# Autodesk Inventor assembly: BBM Staging Plate Assembly
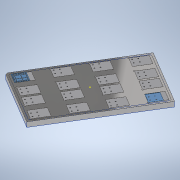
[picture p0: Inventor's stored thumbnail of the model, 180x180]
Saved by Autodesk Inventor 2022 (Build 260153000, 153)
## iProperties
Created: 2021-01-11
Part Number: BBM Staging Plate Assembly
Document SubType Name: Assembly
Designer: caleb
Author: caleb
## Documents named in this file (5)
- C:\Users\Caleb\Desktop\nebraska-silicon-lab\Hardware\ETL\Module Assembly\BBM Staging Plate - V2\BBM Staging Plate Assembly - V2.iam
- C:\Users\Caleb\Desktop\nebraska-silicon-lab\Hardware\ETL\Module Assembly\BBM Staging Plate - V2\BBM Staging Plate - V2.ipt
- C:\Users\Caleb\Desktop\nebraska-silicon-lab\Hardware\ETL\Module Assembly\BBM Staging Plate - V2\BBM Staging Plate Stencil - V2.ipt
- C:\Users\Caleb\Desktop\nebraska-silicon-lab\Hardware\ETL\Module Assembly\BBM Staging Plate - V2\Plastic Inlay.ipt
- C:\Users\Caleb\Desktop\nebraska-silicon-lab\Hardware\ETL\Module Assembly\BBM Staging Plate - V2\F10112319--_1-MODULE_ CMS2 ETL_ PIXEL SENSOR READOUT CHIP.ipt
## Components (5 placed, 4 different names)
1. BBM Staging Plate - V2:1 — Flush:1, Flush:2, Mate:1, Mate:2, Mate:3, Mate:4
2. BBM Staging Plate Stencil - V2:1 — Flush:1, Flush:2, Mate:1, Mate:6, Mate:7, Mate:9, Mate:10
3. Plastic Inlay:1 — Mate:2, Mate:3, Mate:4, Mate:5, Mate:8
4. F10112319--_1-MODULE_ CMS2 ETL_ PIXEL SENSOR READOUT CHIP:1 — Mate:5, Mate:6, Mate:7
5. F10112319--_1-MODULE_ CMS2 ETL_ PIXEL SENSOR READOUT CHIP:2 — Mate:8, Mate:9, Mate:10
## Relationships (12: Mate 10, Flush 2)
- Flush:1: BBM Staging Plate - V2:1 ↔ BBM Staging Plate Stencil - V2:1
- Flush:2: BBM Staging Plate - V2:1 ↔ BBM Staging Plate Stencil - V2:1
- Mate:1: BBM Staging Plate - V2:1 ↔ BBM Staging Plate Stencil - V2:1
- Mate:2: BBM Staging Plate - V2:1 ↔ Plastic Inlay:1
- Mate:3: BBM Staging Plate - V2:1 ↔ Plastic Inlay:1
- Mate:4: BBM Staging Plate - V2:1 ↔ Plastic Inlay:1
- Mate:5: Plastic Inlay:1 ↔ F10112319--_1-MODULE_ CMS2 ETL_ PIXEL SENSOR READOUT CHIP:1
- Mate:6: BBM Staging Plate Stencil - V2:1 ↔ F10112319--_1-MODULE_ CMS2 ETL_ PIXEL SENSOR READOUT CHIP:1
- Mate:7: BBM Staging Plate Stencil - V2:1 ↔ F10112319--_1-MODULE_ CMS2 ETL_ PIXEL SENSOR READOUT CHIP:1
- Mate:8: Plastic Inlay:1 ↔ F10112319--_1-MODULE_ CMS2 ETL_ PIXEL SENSOR READOUT CHIP:2
- Mate:9: BBM Staging Plate Stencil - V2:1 ↔ F10112319--_1-MODULE_ CMS2 ETL_ PIXEL SENSOR READOUT CHIP:2
- Mate:10: BBM Staging Plate Stencil - V2:1 ↔ F10112319--_1-MODULE_ CMS2 ETL_ PIXEL SENSOR READOUT CHIP:2
